# Autodesk Inventor assembly: Custom Cover v0.3
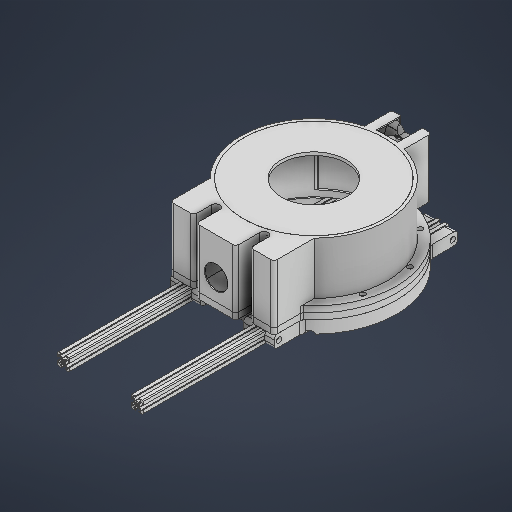
[picture p0: Inventor's stored thumbnail of the model, 512x512]
Saved by Autodesk Inventor 2025 (Build 290162000, 162)
## iProperties
Created: 2024-10-25
Part Number: Custom Cover v0.3
Document SubType Name: Assembly
Designer: mayhe
Author: mayhe
## Documents named in this file (13)
- C:\Users\mayhe\OneDrive\Documents\GitHub\In-situ-monitoring-of-powder-bed-fusion-additive-manufacturing\system_development\Orichalcum\v0.2\Hardware_design\custom-cover\Custom Cover v0.3.iam
- C:\Users\mayhe\OneDrive\Documents\GitHub\In-situ-monitoring-of-powder-bed-fusion-additive-manufacturing\system_development\Orichalcum\v0.2\Hardware_design\custom-cover\cover\Updated Cover.ipt
- C:\Users\mayhe\OneDrive\Documents\GitHub\In-situ-monitoring-of-powder-bed-fusion-additive-manufacturing\system_development\Orichalcum\v0.2\Hardware_design\custom-cover\cylinder-parts\Cylinder 80-20 Spacer_2.ipt
- C:\Users\mayhe\OneDrive\Documents\GitHub\In-situ-monitoring-of-powder-bed-fusion-additive-manufacturing\system_development\Orichalcum\v0.2\Hardware_design\custom-cover\cylinder-parts\Cylinder 80-20 Spacer_1.ipt
- C:\Users\mayhe\OneDrive\Documents\GitHub\In-situ-monitoring-of-powder-bed-fusion-additive-manufacturing\system_development\Orichalcum\v0.2\Hardware_design\custom-cover\8020-parts\20-2020-500-CL.ipt
- C:\Users\mayhe\OneDrive\Documents\GitHub\In-situ-monitoring-of-powder-bed-fusion-additive-manufacturing\system_development\Orichalcum\v0.2\Hardware_design\custom-cover\cylinder-parts\Cylinder 80-20 Spacer_1 Slant.ipt
- C:\Users\mayhe\OneDrive\Documents\GitHub\In-situ-monitoring-of-powder-bed-fusion-additive-manufacturing\system_development\Orichalcum\v0.2\Hardware_design\Full Printer Assembly\Printer Body v6.ipt
- C:\Users\mayhe\OneDrive\Documents\GitHub\In-situ-monitoring-of-powder-bed-fusion-additive-manufacturing\system_development\Orichalcum\v0.2\Hardware_design\custom-cover\cylinder-parts\final-parts\Cylinder Bottom Ring.ipt
- C:\Users\mayhe\OneDrive\Documents\GitHub\In-situ-monitoring-of-powder-bed-fusion-additive-manufacturing\system_development\Orichalcum\v0.2\Hardware_design\custom-cover\cylinder-parts\Cylinder 80-20 Spacer_2 cable hole.ipt
- C:\Users\mayhe\OneDrive\Documents\GitHub\In-situ-monitoring-of-powder-bed-fusion-additive-manufacturing\system_development\Orichalcum\v0.2\Hardware_design\custom-cover\cylinder-parts\final-parts\Cylinder Slidey Bit Housing Camera + galvo.ipt
- C:\Users\mayhe\OneDrive\Documents\GitHub\In-situ-monitoring-of-powder-bed-fusion-additive-manufacturing\system_development\Orichalcum\v0.2\Hardware_design\custom-cover\cylinder-parts\cylinder-segments\Cylinder Segment  Camera + Galvo.ipt
- C:\Users\mayhe\OneDrive\Documents\GitHub\In-situ-monitoring-of-powder-bed-fusion-additive-manufacturing\system_development\Orichalcum\v0.2\Hardware_design\optical-camera\flircamera+lens.ipt
- C:\Users\mayhe\OneDrive\Documents\GitHub\In-situ-monitoring-of-powder-bed-fusion-additive-manufacturing\system_development\Orichalcum\v0.2\Hardware_design\pzt-parts\substrate plate.ipt
## Components (13 placed, 12 different names)
1. Updated Cover:1 — Mate:49, Mate:50, Mate:51, Rotational:8
2. Printer Body v6:1 — Mate:49, Mate:50, Mate:51, Rotational:15
3. Cylinder Bottom Ring:1 — Rotational:8, Rotational:9, Rotational:10, Rotational:11, Mate:52, Mate:54, Mate:56, Mate:58
4. Cylinder 80-20 Spacer_2 cable hole:1 — Rotational:11
5. Cylinder 80-20 Spacer_2:1 — Rotational:10, Rotational:12, Mate:59
6. Cylinder 80-20 Spacer_1 Slant:1 — Mate:56, Mate:57, Mate:58
7. Cylinder 80-20 Spacer_1:1 — Rotational:9, Flush:1, Mate:53, Flush:2, Mate:55
8. 20-2020-500-CL:1 — Mate:52, Flush:1, Mate:53
9. 20-2020-500-CL:2 — Mate:54, Flush:2, Mate:55, Mate:57
10. Cylinder Slidey Bit Housing Camera + galvo:1 — Rotational:13, Mate:60, Rotational:14
11. Cylinder Segment  Camera + Galvo:1 — Rotational:12, Mate:59, Rotational:13, Mate:60
12. flircamera+lens:1 — Rotational:14
13. substrate plate:2 — Rotational:15
## Relationships (22: Mate 12, RevoluteJoint 8, Flush 2)
- Mate:49: Updated Cover:1 ↔ Printer Body v6:1
- Mate:50: Updated Cover:1 ↔ Printer Body v6:1
- Mate:51: Updated Cover:1 ↔ Printer Body v6:1
- Rotational:8 [RevoluteJoint]: Updated Cover:1 ↔ Cylinder Bottom Ring:1
- Rotational:9 [RevoluteJoint]: Cylinder Bottom Ring:1 ↔ Cylinder 80-20 Spacer_1:1
- Rotational:10 [RevoluteJoint]: Cylinder Bottom Ring:1 ↔ Cylinder 80-20 Spacer_2:1
- Rotational:11 [RevoluteJoint]: Cylinder Bottom Ring:1 ↔ Cylinder 80-20 Spacer_2 cable hole:1
- Mate:52: Cylinder Bottom Ring:1 ↔ 20-2020-500-CL:1
- Flush:1: Cylinder 80-20 Spacer_1:1 ↔ 20-2020-500-CL:1
- Mate:53: Cylinder 80-20 Spacer_1:1 ↔ 20-2020-500-CL:1
- Mate:54: Cylinder Bottom Ring:1 ↔ 20-2020-500-CL:2
- Flush:2: Cylinder 80-20 Spacer_1:1 ↔ 20-2020-500-CL:2
- Mate:55: Cylinder 80-20 Spacer_1:1 ↔ 20-2020-500-CL:2
- Mate:56: Cylinder Bottom Ring:1 ↔ Cylinder 80-20 Spacer_1 Slant:1
- Mate:57: Cylinder 80-20 Spacer_1 Slant:1 ↔ 20-2020-500-CL:2
- Mate:58: Cylinder Bottom Ring:1 ↔ Cylinder 80-20 Spacer_1 Slant:1
- Rotational:12 [RevoluteJoint]: Cylinder 80-20 Spacer_2:1 ↔ Cylinder Segment  Camera + Galvo:1
- Mate:59: Cylinder 80-20 Spacer_2:1 ↔ Cylinder Segment  Camera + Galvo:1
- Rotational:13 [RevoluteJoint]: Cylinder Slidey Bit Housing Camera + galvo:1 ↔ Cylinder Segment  Camera + Galvo:1
- Mate:60: Cylinder Slidey Bit Housing Camera + galvo:1 ↔ Cylinder Segment  Camera + Galvo:1
- Rotational:14 [RevoluteJoint]: Cylinder Slidey Bit Housing Camera + galvo:1 ↔ flircamera+lens:1
- Rotational:15 [RevoluteJoint]: Printer Body v6:1 ↔ substrate plate:2
